# Autodesk Inventor assembly: GetriebeC
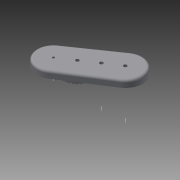
[picture p0: Inventor's stored thumbnail of the model, 180x180]
Saved by Autodesk Inventor 2014 (Build 180170000, 170)
## iProperties
Created: 2013-05-31
Part Number: GetriebeC
Document SubType Name: Assembly
Designer: hanse
Author: hanse
## Documents named in this file (6)
- C:\Users\hanse\Desktop\Beep\Hardware\GetriebeB\GetriebeC.iam
- C:\Users\hanse\Desktop\Beep\Hardware\GetriebeB\DoppelZahnrad.iam
- C:\Users\hanse\Desktop\Beep\Hardware\GetriebeB\Gertiebe\Konstruktions-Assistent\Stirnräder3.iam
- C:\Users\hanse\Desktop\Beep\Hardware\GetriebeB\BFront.ipt
- C:\Users\hanse\Desktop\Beep\Hardware\GetriebeB\EncoderWheel2.ipt
- C:\Users\hanse\Desktop\Beep\Hardware\EE-SX1131.ipt
## Components (7 placed, 5 different names)
1. Stirnräder:1 [sub-assembly] — Passend:8
2. DoppelZahnrad:1 [sub-assembly] — Passend:2, Passend:9
3. DoppelZahnrad:2 [sub-assembly] — Passend:2, Passend:3, Passend:10
4. DoppelZahnrad:3 [sub-assembly] — Passend:3, Passend:11
5. BFront:1
6. EncoderWheel2:1 — Passend:12, Passend:13
7. EE-SX1131:1 — Passend:12
## Relationships (8: Mate 8)
- Passend:2 [Mate] (15 mm): DoppelZahnrad:1 ↔ DoppelZahnrad:2
- Passend:3 [Mate] (15 mm): DoppelZahnrad:2 ↔ DoppelZahnrad:3
- Passend:8 [Mate]: Stirnräder:1
- Passend:9 [Mate]: DoppelZahnrad:1
- Passend:10 [Mate]: DoppelZahnrad:2
- Passend:11 [Mate]: DoppelZahnrad:3
- Passend:12 [Mate] (0.1 mm): EncoderWheel2:1 ↔ EE-SX1131:1
- Passend:13 [Mate]: EncoderWheel2:1
